# Autodesk Inventor assembly: head_mind
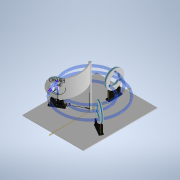
[picture p0: Inventor's stored thumbnail of the model, 180x180]
Saved by Autodesk Inventor 2021.1 (Build 251245010, 245A)
## iProperties
Created: 2023-01-21
Part Number: head_mind
Document SubType Name: Assembly
Designer: zmoze
Author: zmoze
## Documents named in this file (6)
- C:\Users\zmoze\OneDrive\Рабочий стол\GrabCAD\Smile_2022-2023\head_mind.iam
- C:\Users\zmoze\OneDrive\Рабочий стол\GrabCAD\Smile_2022-2023\держалка_мозговорота.iam
- C:\Users\zmoze\OneDrive\Рабочий стол\GrabCAD\Smile_2022-2023\верхняя пластина.ipt
- C:\Users\zmoze\OneDrive\Рабочий стол\GrabCAD\Smile_2022-2023\трубочки_мозговорота.ipt
- C:\Users\zmoze\OneDrive\Рабочий стол\GrabCAD\Smile_2022-2023\шаговый_мотор.ipt
- C:\Users\zmoze\OneDrive\Рабочий стол\GrabCAD\Smile_2022-2023\локатор.ipt
## Components (7 placed, 5 different names)
1. верхняя пластина:1 — Совмещение:1, Заподлицо:1, Совмещение:2, Совмещение:3, Совмещение:5, Совмещение:7
2. трубочки_мозговорота:1 — Совмещение:3, Совмещение:4, Совмещение:6
3. шаговый_мотор:1 — Совмещение:5, Совмещение:6, Совмещение:7, Совмещение:8, Совмещение:9
4. локатор:1 — Совмещение:8, Совмещение:9
5. держалка_мозговорота:1 [sub-assembly] — Совмещение:1, Заподлицо:1, Совмещение:2
6. держалка_мозговорота:2 [sub-assembly] — Совмещение:4
7. держалка_мозговорота:3 [sub-assembly]
## Component patterns: (3 elements, first: держалка_мозговорота:1)
## Relationships (10: Mate 9, Flush 1)
- Совмещение:1 [Mate]: верхняя пластина:1 ↔ держалка_мозговорота:1
- Заподлицо:1 [Flush] (25 mm): верхняя пластина:1 ↔ держалка_мозговорота:1
- Совмещение:2 [Mate]: верхняя пластина:1 ↔ держалка_мозговорота:1
- Совмещение:3 [Mate]: верхняя пластина:1 ↔ трубочки_мозговорота:1
- Совмещение:4 [Mate]: трубочки_мозговорота:1 ↔ держалка_мозговорота:2
- Совмещение:5 [Mate]: верхняя пластина:1 ↔ шаговый_мотор:1
- Совмещение:6 [Mate]: трубочки_мозговорота:1 ↔ шаговый_мотор:1
- Совмещение:7 [Mate]: верхняя пластина:1 ↔ шаговый_мотор:1
- Совмещение:8 [Mate]: шаговый_мотор:1 ↔ локатор:1
- Совмещение:9 [Mate]: шаговый_мотор:1 ↔ локатор:1
